# Autodesk Inventor assembly: mobile
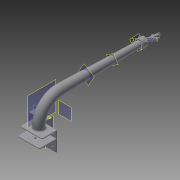
[picture p0: Inventor's stored thumbnail of the model, 180x180]
Saved by Autodesk Inventor 2014 (Build 180170000, 170)
## iProperties
Created: 2017-08-03
Part Number: mobile
Document SubType Name: Assembly
Designer: hide
Author: hide
## Documents named in this file (11)
- Z:\src\github.com\stem-dad\diy-baby-crib-mobile\models\mobile.iam
- Z:\src\github.com\stem-dad\diy-baby-crib-mobile\models\pole-bottom.ipt
- Z:\src\github.com\stem-dad\diy-baby-crib-mobile\models\pole-center.ipt
- Z:\src\github.com\stem-dad\diy-baby-crib-mobile\models\pole-top.ipt
- Z:\src\github.com\stem-dad\diy-baby-crib-mobile\models\stick-holder-top2.ipt
- Z:\src\github.com\stem-dad\diy-baby-crib-mobile\models\top-star.ipt
- Z:\src\github.com\stem-dad\diy-baby-crib-mobile\models\motor-holder.ipt
- Z:\src\github.com\stem-dad\diy-baby-crib-mobile\models\pole-corner.ipt
- Z:\src\github.com\stem-dad\diy-baby-crib-mobile\models\bed-stopper.ipt
- Z:\src\github.com\stem-dad\diy-baby-crib-mobile\models\arduino-holder.ipt
- Z:\src\github.com\stem-dad\diy-baby-crib-mobile\models\arduino-holder-cover.ipt
## Components (10 placed, 10 different names)
1. pole-bottom:1 — メイト:1, メイト:2, メイト:3, メイト:14, メイト:15, メイト:19
2. pole-center:1 — メイト:1, メイト:2, メイト:3, メイト:4, メイト:5, メイト:6
3. pole-top:1 — メイト:4, メイト:5, メイト:6, メイト:11, メイト:12, メイト:21
4. stick-holder-top2:1 — メイト:7, メイト:8, メイト:9, メイト:10, 角度:1
5. top-star:1 — メイト:9, メイト:10, 角度:1
6. motor-holder:1 — メイト:7, メイト:8, メイト:11, メイト:12, メイト:21
7. pole-corner:1 — メイト:14, メイト:15, メイト:17, メイト:18, メイト:19, メイト:20
8. bed-stopper:1 — メイト:17, メイト:18, メイト:20, メイト:22, メイト:23, メイト:24
9. arduino-holder:1 — メイト:22, メイト:23, メイト:24, メイト:25, メイト:26, メイト:27
10. arduino-holder-cover:1 — メイト:25, メイト:26, メイト:27
## Relationships (26: Mate 25, Angle 1)
- メイト:1 [Mate]: pole-bottom:1 ↔ pole-center:1
- メイト:2 [Mate]: pole-bottom:1 ↔ pole-center:1
- メイト:3 [Mate]: pole-bottom:1 ↔ pole-center:1
- メイト:4 [Mate]: pole-center:1 ↔ pole-top:1
- メイト:5 [Mate]: pole-center:1 ↔ pole-top:1
- メイト:6 [Mate]: pole-center:1 ↔ pole-top:1
- メイト:7 [Mate]: stick-holder-top2:1 ↔ motor-holder:1
- メイト:8 [Mate] (1 mm): stick-holder-top2:1 ↔ motor-holder:1
- メイト:9 [Mate]: stick-holder-top2:1 ↔ top-star:1
- メイト:10 [Mate]: stick-holder-top2:1 ↔ top-star:1
- 角度:1 [Angle] (0 deg): stick-holder-top2:1 ↔ top-star:1
- メイト:11 [Mate]: pole-top:1 ↔ motor-holder:1
- メイト:12 [Mate]: pole-top:1 ↔ motor-holder:1
- メイト:14 [Mate]: pole-bottom:1 ↔ pole-corner:1
- メイト:15 [Mate]: pole-bottom:1 ↔ pole-corner:1
- メイト:17 [Mate]: pole-corner:1 ↔ bed-stopper:1
- メイト:18 [Mate]: pole-corner:1 ↔ bed-stopper:1
- メイト:19 [Mate]: pole-bottom:1 ↔ pole-corner:1
- メイト:20 [Mate]: pole-corner:1 ↔ bed-stopper:1
- メイト:21 [Mate]: pole-top:1 ↔ motor-holder:1
- メイト:22 [Mate]: bed-stopper:1 ↔ arduino-holder:1
- メイト:23 [Mate]: bed-stopper:1 ↔ arduino-holder:1
- メイト:24 [Mate]: bed-stopper:1 ↔ arduino-holder:1
- メイト:25 [Mate]: arduino-holder:1 ↔ arduino-holder-cover:1
- メイト:26 [Mate]: arduino-holder:1 ↔ arduino-holder-cover:1
- メイト:27 [Mate]: arduino-holder:1 ↔ arduino-holder-cover:1
